# Autodesk Inventor assembly: cnc motor support
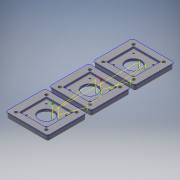
[picture p0: Inventor's stored thumbnail of the model, 180x180]
Saved by Autodesk Inventor 2016 SP1 (Build 200210100, 210)
## iProperties
Created: 2016-04-15
Part Number: cnc motor support
Document SubType Name: Assembly
Designer: ubik
Author: ubik
## Documents named in this file (2)
- E:\GitHub\kossel-XXL\cnc motor support.iam
- E:\GitHub\kossel-XXL\motor support.ipt
## Components (3 placed, 1 different names)
1. motor support:1 — Mate:1, Flush:1, Flush:2
2. motor support:2 — Mate:1, Mate:2, Flush:1, Flush:2, Flush:3, Flush:4
3. motor support:3 — Mate:2, Flush:3, Flush:4
## Relationships (6: Flush 4, Mate 2)
- Mate:1 (8 mm): motor support:1 ↔ motor support:2
- Mate:2 (8 mm): motor support:2 ↔ motor support:3
- Flush:1: motor support:1 ↔ motor support:2
- Flush:2: motor support:1 ↔ motor support:2
- Flush:3: motor support:2 ↔ motor support:3
- Flush:4: motor support:2 ↔ motor support:3
